# Autodesk Inventor assembly: rovPrototype1
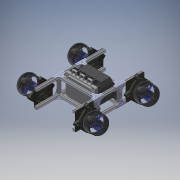
[picture p0: Inventor's stored thumbnail of the model, 180x180]
Saved by Autodesk Inventor 2018 (Build 220112000, 112)
## iProperties
Created: 2019-02-03
Part Number: rovPrototype1
Document SubType Name: Assembly
Designer: anirudh
Author: anirudh
## Documents named in this file (10)
- C:\Users\anirudh\Documents\MARS Fund\MATE Robotics\Silicon Sharks\2018-2019\rovPrototype1.iam
- C:\Users\anirudh\Documents\MARS Fund\MATE Robotics\Silicon Sharks\2018-2019\15inREV.ipt
- C:\Users\anirudh\Documents\MARS Fund\MATE Robotics\Silicon Sharks\2018-2019\12inREV.ipt
- C:\Users\anirudh\Documents\MARS Fund\MATE Robotics\Silicon Sharks\2018-2019\4inREV.ipt
- C:\Users\anirudh\Downloads\REV-41-1025.ipt
- C:\Users\anirudh\Documents\MARS Fund\MATE Robotics\Silicon Sharks\2018-2019\LazySusanBearing.ipt
- C:\Users\anirudh\Documents\MARS Fund\MATE Robotics\Silicon Sharks\2018-2019\ThrusterMount.ipt
- C:\Users\anirudh\Documents\MARS Fund\MATE Robotics\Silicon Sharks\2018-2019\T200-THRUSTER-R1.ipt
- C:\Users\anirudh\Documents\MARS Fund\MATE Robotics\Silicon Sharks\2018-2019\ElectronicsHousing.iam
- C:\Users\anirudh\Downloads\REV-41-1039.ipt
## Components (45 placed, 9 different names)
1. 15inREV:1 — Flush:3, Flush:4, Mate:2, Flush:5, Flush:6, Mate:3, Mate:5, Mate:6, Flush:12, Flush:19, Flush:21, Mate:16, Mate:17, Flush:33, Flush:34, Mate:20, Mate:21, Flush:39, Flush:41, Symmetry:1, Mate:51, Flush:71, Flush:72, Mate:52, Flush:73, Flush:74, Flush:79
2. 15inREV:2 — Flush:3, Flush:4, Mate:2, Flush:14, Mate:10, Mate:11, Mate:18, Mate:19, Flush:35, Flush:36, Mate:22, Mate:23, Flush:45, Flush:46
3. 15inREV:3 — Flush:1, Flush:2, Mate:1, Flush:5, Flush:6, Mate:3, Mate:4, Flush:7, Flush:11, Mate:7, Flush:15, Flush:17, Flush:23, Mate:12, Flush:25, Mate:24, Flush:47, Flush:49, Mate:25, Mate:26, Mate:27, Symmetry:1, Mate:47, Mate:55, Flush:80, Flush:81, Mate:56, Flush:82, Flush:83
4. 15inREV:4 — Flush:1, Flush:2, Mate:1, Flush:10, Mate:8, Mate:9, Mate:14, Mate:15, Flush:27, Flush:29, Flush:53, Flush:54
5. 12inREV:1 — Flush:13, Mate:7, Flush:14, Flush:30, Flush:37, Flush:66, Mate:44
6. 12inREV:2 — Flush:11, Mate:6, Flush:12, Flush:13, Flush:18, Flush:22, Mate:13, Flush:26, Flush:31, Mate:42, Flush:65, Mate:46, Flush:67, Mate:49
7. 12inREV:3 — Flush:9, Mate:5, Flush:10, Flush:28, Flush:38
8. 12inREV:4 — Mate:4, Flush:7, Flush:9, Flush:16, Flush:20, Flush:24, Flush:32, Flush:79
9. 4inREV:1 — Flush:15, Flush:16, Mate:8, Flush:50, Flush:52
10. 4inREV:2 — Flush:21, Flush:22, Mate:11, Flush:40, Flush:43, Mate:43, Flush:68
11. 4inREV:3 — Flush:17, Flush:18, Mate:9, Flush:48, Flush:51, Mate:45, Mate:50
12. 4inREV:4 — Flush:19, Flush:20, Mate:10, Flush:42, Flush:44
13. REV-41-1025:1 — Mate:14, Flush:29, Flush:30
14. REV-41-1025:2 — Flush:23, Flush:24, Mate:12
15. REV-41-1025:3 — Mate:15, Flush:27, Flush:28
16. REV-41-1025:4 — Mate:13, Flush:25, Flush:26
17. REV-41-1025:5 — Mate:18, Flush:35, Flush:38
18. REV-41-1025:6 — Mate:19, Flush:36, Flush:37
19. REV-41-1025:7 — Mate:17, Flush:31, Flush:34
20. REV-41-1025:8 — Mate:16, Flush:32, Flush:33
21. REV-41-1025:9 — Mate:27, Flush:51, Flush:53
22. REV-41-1025:10 — Flush:49, Mate:25, Flush:50
23. REV-41-1025:11 — Mate:24, Flush:47, Flush:48
24. REV-41-1025:12 — Mate:26, Flush:52, Flush:54
25. REV-41-1025:13 — Mate:20, Flush:41, Flush:42
26. REV-41-1025:14 — Mate:21, Flush:39, Flush:40
27. REV-41-1025:15 — Mate:23, Flush:43, Flush:46
28. REV-41-1025:16 — Mate:22, Flush:44, Flush:45
29. ElectronicsHousing:1 [sub-assembly] — Mate:46, Mate:47, Flush:67
30. 4inREV:5 — Mate:42, Mate:43, Flush:65, Mate:48
31. 4inREV:6 — Flush:66, Mate:44, Mate:45, Flush:69
32. REV-41-1039:1 — Mate:48, Flush:68, Mate:49, Flush:70
33. REV-41-1039:2 — Mate:50, Flush:69, Flush:70
34. LazySusanBearing:1 — Mate:51, Flush:71, Flush:72, Mate:53, Flush:75, Flush:76
35. LazySusanBearing:2 — Mate:52, Flush:73, Flush:74, Mate:54, Flush:77, Flush:78
36. ThrusterMount:1 — Mate:53, Flush:75, Flush:76, Mate:59, Mate:60, Mate:61
37. ThrusterMount:2 — Mate:54, Flush:77, Flush:78, Mate:62, Mate:63, Mate:64
38. LazySusanBearing:3 — Mate:55, Flush:80, Flush:81, Mate:57, Flush:84, Flush:86
39. LazySusanBearing:4 — Mate:56, Flush:82, Flush:83, Mate:58, Flush:85, Flush:87
40. ThrusterMount:3 — Mate:57, Flush:85, Flush:87, Mate:66, Mate:67, Mate:68
41. ThrusterMount:4 — Mate:58, Flush:84, Flush:86, Mate:65, Mate:69, Mate:70
42. T200-THRUSTER-R1:1 — Mate:59, Mate:60, Mate:61
43. T200-THRUSTER-R1:2 — Mate:62, Mate:63, Mate:64
44. T200-THRUSTER-R1:3 — Mate:65, Mate:69, Mate:70
45. T200-THRUSTER-R1:4 — Mate:66, Mate:67, Mate:68
## Relationships (133: Flush 76, Mate 56, Symmetry 1)
- Flush:1: 15inREV:3 ↔ 15inREV:4
- Flush:2: 15inREV:3 ↔ 15inREV:4
- Mate:1 (71.6 mm): 15inREV:3 ↔ 15inREV:4
- Flush:3: 15inREV:1 ↔ 15inREV:2
- Flush:4: 15inREV:1 ↔ 15inREV:2
- Mate:2 (71.6 mm): 15inREV:1 ↔ 15inREV:2
- Flush:5: 15inREV:1 ↔ 15inREV:3
- Flush:6: 15inREV:1 ↔ 15inREV:3
- Mate:3 (195.263 mm): 15inREV:1 ↔ 15inREV:3
- Mate:4: 15inREV:3 ↔ 12inREV:4
- Flush:7: 15inREV:3 ↔ 12inREV:4
- Flush:9: 12inREV:3 ↔ 12inREV:4
- Mate:5: 15inREV:1 ↔ 12inREV:3
- Flush:10: 15inREV:4 ↔ 12inREV:3
- Flush:11: 15inREV:3 ↔ 12inREV:2
- Mate:6: 15inREV:1 ↔ 12inREV:2
- Flush:12 (-121.5898 mm): 15inREV:1 ↔ 12inREV:2
- Flush:13: 12inREV:1 ↔ 12inREV:2
- Mate:7: 15inREV:3 ↔ 12inREV:1
- Flush:14: 15inREV:2 ↔ 12inREV:1
- Flush:15: 15inREV:3 ↔ 4inREV:1
- Flush:16: 12inREV:4 ↔ 4inREV:1
- Mate:8: 15inREV:4 ↔ 4inREV:1
- Flush:17: 15inREV:3 ↔ 4inREV:3
- Flush:18: 12inREV:2 ↔ 4inREV:3
- Mate:9: 15inREV:4 ↔ 4inREV:3
- Flush:19: 15inREV:1 ↔ 4inREV:4
- Flush:20: 12inREV:4 ↔ 4inREV:4
- Mate:10: 15inREV:2 ↔ 4inREV:4
- Flush:21: 15inREV:1 ↔ 4inREV:2
- Flush:22: 12inREV:2 ↔ 4inREV:2
- Mate:11: 15inREV:2 ↔ 4inREV:2
- Flush:23: 15inREV:3 ↔ REV-41-1025:2
- Flush:24: 12inREV:4 ↔ REV-41-1025:2
- Mate:12: 15inREV:3 ↔ REV-41-1025:2
- Mate:13: 12inREV:2 ↔ REV-41-1025:4
- Flush:25: 15inREV:3 ↔ REV-41-1025:4
- Flush:26: 12inREV:2 ↔ REV-41-1025:4
- Mate:14: 15inREV:4 ↔ REV-41-1025:1
- Mate:15: 15inREV:4 ↔ REV-41-1025:3
- Flush:27: 15inREV:4 ↔ REV-41-1025:3
- Flush:28: 12inREV:3 ↔ REV-41-1025:3
- Flush:29: 15inREV:4 ↔ REV-41-1025:1
- Flush:30: 12inREV:1 ↔ REV-41-1025:1
- Mate:16: 15inREV:1 ↔ REV-41-1025:8
- Mate:17: 15inREV:1 ↔ REV-41-1025:7
- Flush:31: 12inREV:2 ↔ REV-41-1025:7
- Flush:32: 12inREV:4 ↔ REV-41-1025:8
- Flush:33: 15inREV:1 ↔ REV-41-1025:8
- Flush:34: 15inREV:1 ↔ REV-41-1025:7
- Mate:18: 15inREV:2 ↔ REV-41-1025:5
- Mate:19: 15inREV:2 ↔ REV-41-1025:6
- Flush:35: 15inREV:2 ↔ REV-41-1025:5
- Flush:36: 15inREV:2 ↔ REV-41-1025:6
- Flush:37: 12inREV:1 ↔ REV-41-1025:6
- Flush:38: 12inREV:3 ↔ REV-41-1025:5
- Mate:20: 15inREV:1 ↔ REV-41-1025:13
- Mate:21: 15inREV:1 ↔ REV-41-1025:14
- Flush:39: 15inREV:1 ↔ REV-41-1025:14
- Flush:40: 4inREV:2 ↔ REV-41-1025:14
- Flush:41: 15inREV:1 ↔ REV-41-1025:13
- Flush:42: 4inREV:4 ↔ REV-41-1025:13
- Mate:22: 15inREV:2 ↔ REV-41-1025:16
- Mate:23: 15inREV:2 ↔ REV-41-1025:15
- Flush:43: 4inREV:2 ↔ REV-41-1025:15
- Flush:44: 4inREV:4 ↔ REV-41-1025:16
- Flush:45: 15inREV:2 ↔ REV-41-1025:16
- Flush:46: 15inREV:2 ↔ REV-41-1025:15
- Mate:24: 15inREV:3 ↔ REV-41-1025:11
- Flush:47: 15inREV:3 ↔ REV-41-1025:11
- Flush:48: 4inREV:3 ↔ REV-41-1025:11
- Flush:49: 15inREV:3 ↔ REV-41-1025:10
- Mate:25: 15inREV:3 ↔ REV-41-1025:10
- Flush:50: 4inREV:1 ↔ REV-41-1025:10
- Mate:26: 15inREV:3 ↔ REV-41-1025:12
- Mate:27: 15inREV:3 ↔ REV-41-1025:9
- Flush:51: 4inREV:3 ↔ REV-41-1025:9
- Flush:52: 4inREV:1 ↔ REV-41-1025:12
- Flush:53: 15inREV:4 ↔ REV-41-1025:9
- Flush:54: 15inREV:4 ↔ REV-41-1025:12
- Symmetry:1: 15inREV:1 ↔ 15inREV:3
- Mate:42: 12inREV:2 ↔ 4inREV:5
- Mate:43: 4inREV:2 ↔ 4inREV:5
- Flush:65: 12inREV:2 ↔ 4inREV:5
- Flush:66: 12inREV:1 ↔ 4inREV:6
- Mate:44: 12inREV:1 ↔ 4inREV:6
- Mate:45: 4inREV:3 ↔ 4inREV:6
- Mate:46: 12inREV:2 ↔ ElectronicsHousing:1
- Mate:47: 15inREV:3 ↔ ElectronicsHousing:1
- Flush:67: 12inREV:2 ↔ ElectronicsHousing:1
- Mate:48: 4inREV:5 ↔ REV-41-1039:1
- Flush:68: 4inREV:2 ↔ REV-41-1039:1
- Mate:49 (15.7988 mm): 12inREV:2 ↔ REV-41-1039:1
- Mate:50: 4inREV:3 ↔ REV-41-1039:2
- Flush:69: 4inREV:6 ↔ REV-41-1039:2
- Flush:70: REV-41-1039:1 ↔ REV-41-1039:2
- Mate:51: 15inREV:1 ↔ LazySusanBearing:1
- Flush:71: 15inREV:1 ↔ LazySusanBearing:1
- Flush:72: 15inREV:1 ↔ LazySusanBearing:1
- Mate:52: 15inREV:1 ↔ LazySusanBearing:2
- Flush:73: 15inREV:1 ↔ LazySusanBearing:2
- Flush:74: 15inREV:1 ↔ LazySusanBearing:2
- Mate:53: LazySusanBearing:1 ↔ ThrusterMount:1
- Flush:75 (10.3124 mm): LazySusanBearing:1 ↔ ThrusterMount:1
- Flush:76 (10.3124 mm): LazySusanBearing:1 ↔ ThrusterMount:1
- Mate:54: LazySusanBearing:2 ↔ ThrusterMount:2
- Flush:77 (10.3124 mm): LazySusanBearing:2 ↔ ThrusterMount:2
- Flush:78 (10.3124 mm): LazySusanBearing:2 ↔ ThrusterMount:2
- Flush:79 (121.5898 mm): 15inREV:1 ↔ 12inREV:4
- Mate:55: 15inREV:3 ↔ LazySusanBearing:3
- Flush:80: 15inREV:3 ↔ LazySusanBearing:3
- Flush:81: 15inREV:3 ↔ LazySusanBearing:3
- Mate:56: 15inREV:3 ↔ LazySusanBearing:4
- Flush:82: 15inREV:3 ↔ LazySusanBearing:4
- Flush:83: 15inREV:3 ↔ LazySusanBearing:4
- Mate:57: LazySusanBearing:3 ↔ ThrusterMount:3
- Mate:58: LazySusanBearing:4 ↔ ThrusterMount:4
- Flush:84 (10.3124 mm): LazySusanBearing:3 ↔ ThrusterMount:4
- Flush:85 (10.3124 mm): LazySusanBearing:4 ↔ ThrusterMount:3
- Flush:86 (10.3124 mm): LazySusanBearing:3 ↔ ThrusterMount:4
- Flush:87 (10.3124 mm): LazySusanBearing:4 ↔ ThrusterMount:3
- Mate:59: ThrusterMount:1 ↔ T200-THRUSTER-R1:1
- Mate:60: ThrusterMount:1 ↔ T200-THRUSTER-R1:1
- Mate:61: ThrusterMount:1 ↔ T200-THRUSTER-R1:1
- Mate:62: ThrusterMount:2 ↔ T200-THRUSTER-R1:2
- Mate:63: ThrusterMount:2 ↔ T200-THRUSTER-R1:2
- Mate:64: ThrusterMount:2 ↔ T200-THRUSTER-R1:2
- Mate:65: ThrusterMount:4 ↔ T200-THRUSTER-R1:3
- Mate:66: ThrusterMount:3 ↔ T200-THRUSTER-R1:4
- Mate:67: ThrusterMount:3 ↔ T200-THRUSTER-R1:4
- Mate:68: ThrusterMount:3 ↔ T200-THRUSTER-R1:4
- Mate:69: ThrusterMount:4 ↔ T200-THRUSTER-R1:3
- Mate:70: ThrusterMount:4 ↔ T200-THRUSTER-R1:3
